# Autodesk Inventor assembly: POM_T5_01
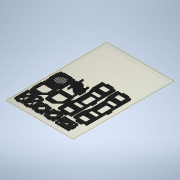
[picture p0: Inventor's stored thumbnail of the model, 180x180]
Saved by Autodesk Inventor 2020 (Build 240168000, 168)
## iProperties
Created: 2021-08-27
Part Number: POM_T5_01
Document SubType Name: Assembly
Designer: Masato
Author: Masato
## Documents named in this file (9)
- C:\Users\aibay\Documents\Inventor\cam\sustaina\OpenPlatform_ver3_0\Cam\POM_T5_01.iam
- C:\Users\aibay\Documents\Inventor\cam\sustaina\OpenPlatform_ver3_0\Cam\DisposableBoard.ipt
- C:\Users\aibay\Documents\Inventor\cam\sustaina\OpenPlatform_ver3_0\UpperBody\Head\Camera_root_frame.ipt
- C:\Users\aibay\Documents\Inventor\cam\sustaina\OpenPlatform_ver3_0\UpperBody\Head\Head_diagonal.ipt
- C:\Users\aibay\Documents\Inventor\cam\sustaina\OpenPlatform_ver3_0\UpperBody\Head\Head_horn_frame.ipt
- C:\Users\aibay\Documents\Inventor\cam\sustaina\OpenPlatform_ver3_0\UpperBody\Arm\ForeArm_diagonal.ipt
- C:\Users\aibay\Documents\Inventor\cam\sustaina\OpenPlatform_ver3_0\UpperBody\Arm\UpperArm_diagonal.ipt
- C:\Users\aibay\Documents\Inventor\cam\sustaina\OpenPlatform_ver3_0\UpperBody\Trunk\Trunk_chest_frame.ipt
- C:\Users\aibay\Documents\Inventor\cam\sustaina\OpenPlatform_ver3_0\UpperBody\Head\Camera_side_frame.ipt
## Components (13 placed, 8 different names)
1. DisposableBoard:1 — メイト:2, メイト:1, フラッシュ:1, フラッシュ:2, フラッシュ:3, フラッシュ:4, メイト:4, メイト:5, メイト:7, メイト:9, メイト:13, メイト:15, メイト:17, メイト:20, メイト:22, メイト:25, メイト:27, メイト:29
2. Camera_root_frame:1 — メイト:27, フラッシュ:11, メイト:28
3. Head_diagonal:1 — フラッシュ:5, メイト:5, メイト:6, メイト:8, メイト:16
4. Head_diagonal:2 — フラッシュ:3, フラッシュ:4, メイト:4, フラッシュ:5, メイト:6, フラッシュ:6, フラッシュ:7, フラッシュ:8, メイト:12, フラッシュ:9, フラッシュ:11
5. Head_horn_frame:1 — メイト:11, フラッシュ:8, メイト:29
6. ForeArm_diagonal:1 — メイト:12, メイト:13, フラッシュ:9, メイト:14, メイト:28
7. ForeArm_diagonal:2 — メイト:14, メイト:15, メイト:16, メイト:18, メイト:23
8. UpperArm_diagonal:1 — メイト:7, メイト:8, フラッシュ:6, メイト:10
9. UpperArm_diagonal:2 — フラッシュ:7, メイト:9, メイト:10, メイト:11, メイト:19
10. Trunk_chest_frame:1 — メイト:17, メイト:18, メイト:19, フラッシュ:10, メイト:21, メイト:24
11. Trunk_chest_frame:2 — フラッシュ:10, メイト:20, メイト:21
12. Camera_side_frame:1 — メイト:25, メイト:26
13. Camera_side_frame:2 — メイト:22, メイト:23, メイト:24, メイト:26
## Relationships (39: Mate 28, Flush 11)
- メイト:2 [Mate]: DisposableBoard:1
- メイト:1 [Mate]: DisposableBoard:1
- フラッシュ:1 [Flush]: DisposableBoard:1
- フラッシュ:2 [Flush]: DisposableBoard:1
- フラッシュ:3 [Flush]: DisposableBoard:1 ↔ Head_diagonal:2
- フラッシュ:4 [Flush]: DisposableBoard:1 ↔ Head_diagonal:2
- メイト:4 [Mate]: DisposableBoard:1 ↔ Head_diagonal:2
- フラッシュ:5 [Flush]: Head_diagonal:1 ↔ Head_diagonal:2
- メイト:5 [Mate]: DisposableBoard:1 ↔ Head_diagonal:1
- メイト:6 [Mate] (2.5 mm): Head_diagonal:1 ↔ Head_diagonal:2
- メイト:7 [Mate]: DisposableBoard:1 ↔ UpperArm_diagonal:1
- メイト:8 [Mate] (2.5 mm): Head_diagonal:1 ↔ UpperArm_diagonal:1
- フラッシュ:6 [Flush]: Head_diagonal:2 ↔ UpperArm_diagonal:1
- フラッシュ:7 [Flush]: Head_diagonal:2 ↔ UpperArm_diagonal:2
- メイト:9 [Mate]: DisposableBoard:1 ↔ UpperArm_diagonal:2
- メイト:10 [Mate] (2.5 mm): UpperArm_diagonal:1 ↔ UpperArm_diagonal:2
- メイト:11 [Mate] (2.5 mm): Head_horn_frame:1 ↔ UpperArm_diagonal:2
- フラッシュ:8 [Flush]: Head_diagonal:2 ↔ Head_horn_frame:1
- メイト:12 [Mate] (2.5 mm): Head_diagonal:2 ↔ ForeArm_diagonal:1
- メイト:13 [Mate]: DisposableBoard:1 ↔ ForeArm_diagonal:1
- フラッシュ:9 [Flush]: Head_diagonal:2 ↔ ForeArm_diagonal:1
- メイト:14 [Mate] (2.5 mm): ForeArm_diagonal:1 ↔ ForeArm_diagonal:2
- メイト:15 [Mate]: DisposableBoard:1 ↔ ForeArm_diagonal:2
- メイト:16 [Mate] (2.5 mm): Head_diagonal:1 ↔ ForeArm_diagonal:2
- メイト:17 [Mate]: DisposableBoard:1 ↔ Trunk_chest_frame:1
- メイト:18 [Mate] (2.5 mm): ForeArm_diagonal:2 ↔ Trunk_chest_frame:1
- メイト:19 [Mate] (2.5 mm): UpperArm_diagonal:2 ↔ Trunk_chest_frame:1
- フラッシュ:10 [Flush]: Trunk_chest_frame:1 ↔ Trunk_chest_frame:2
- メイト:20 [Mate]: DisposableBoard:1 ↔ Trunk_chest_frame:2
- メイト:21 [Mate] (2.5 mm): Trunk_chest_frame:1 ↔ Trunk_chest_frame:2
- メイト:22 [Mate]: DisposableBoard:1 ↔ Camera_side_frame:2
- メイト:23 [Mate] (2.5 mm): ForeArm_diagonal:2 ↔ Camera_side_frame:2
- メイト:24 [Mate] (2.5 mm): Trunk_chest_frame:1 ↔ Camera_side_frame:2
- メイト:25 [Mate]: DisposableBoard:1 ↔ Camera_side_frame:1
- メイト:26 [Mate] (2.5 mm): Camera_side_frame:1 ↔ Camera_side_frame:2
- メイト:27 [Mate]: DisposableBoard:1 ↔ Camera_root_frame:1
- フラッシュ:11 [Flush]: Camera_root_frame:1 ↔ Head_diagonal:2
- メイト:28 [Mate] (2.5 mm): Camera_root_frame:1 ↔ ForeArm_diagonal:1
- メイト:29 [Mate]: DisposableBoard:1 ↔ Head_horn_frame:1
